# Autodesk Inventor assembly: Pancake_Timing Assy_4 Lanes
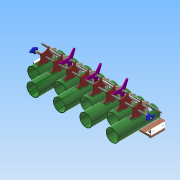
[picture p0: Inventor's stored thumbnail of the model, 180x180]
Saved by Autodesk Inventor 2018.1 (Build 221171000, 171)
## iProperties
Created: 2019-02-11
Part Number: Pancake_Timing Assy_4 Lanes
Document SubType Name: Assembly
Designer: James
Author: James
## Documents named in this file (10)
- C:\Users\admin\Desktop\Ball-Machine\Pancake Sort\Pancake - 4 Lanes\Pancake_Timing Assy_4 Lanes.iam
- C:\Users\admin\Desktop\Ball-Machine\Timing Gate\Nyloc Nut - M4.ipt
- C:\Users\admin\Desktop\Ball-Machine\Timing Gate\Socket Csk Screw - (A2) - M4 x  16.ipt
- C:\Users\admin\Desktop\Ball-Machine\Timing Gate\Socket Cap Screw - Standard - (A2) - M4 x 16.ipt
- C:\Users\admin\Desktop\Ball-Machine\Pancake Sort\Pancake_Angle Bracket.ipt
- C:\Users\admin\Desktop\Ball-Machine\Pancake Sort\Pancake_PVC Pipe.ipt
- C:\Users\admin\Desktop\Ball-Machine\Pancake Sort\Pancake_PVC Pipe Long.ipt
- C:\Users\admin\Desktop\Ball-Machine\Pancake Sort\Pancake - 4 Lanes\Pancake_Timing Assy_Lever Shaft_4 Lanes.iam
- C:\Users\admin\Desktop\Ball-Machine\Pancake Sort\Pancake - 4 Lanes\Pancake_Timing Assy_Star Shaft_4 Lanes.iam
- C:\Users\admin\Desktop\Ball-Machine\Pancake Sort\Pancake - 4 Lanes\Pancake_Timing Backboard_4 Lanes.ipt
## Components (53 placed, 9 different names)
1. Pancake_Timing Backboard_4 Lanes:1 — Angle:2, Tangent:1, Mate:93, Mate:94, Mate:95, Mate:96, Flush:34, Mate:104, Mate:105, Mate:106, Flush:36, Mate:107, Mate:108, Mate:115, Flush:37, Mate:116, Mate:117, Mate:118, Mate:119, Tangent:2, Mate:120, Mate:121
2. Pancake_Timing Assy_Lever Shaft_4 Lanes:1 [sub-assembly] — Flush:96, Flush:97, Flush:31
3. Pancake_Timing Assy_Star Shaft_4 Lanes:1 [sub-assembly] — Flush:94, Angle:2, Flush:93, Flush:95
4. Pancake_Angle Bracket:3 — Mate:104, Mate:105, Mate:106, Flush:36
5. Socket Cap Screw - Standard - (A2) - M4 x 16:7
6. Socket Cap Screw - Standard - (A2) - M4 x 16:8
7. Nyloc Nut - M4:17 — Mate:108
8. Nyloc Nut - M4:18 — Mate:107
9. Pancake_Angle Bracket:4 — Mate:115, Flush:37, Mate:118, Mate:119
10. Nyloc Nut - M4:27 — Mate:117
11. Socket Cap Screw - Standard - (A2) - M4 x 16:9
12. Nyloc Nut - M4:28 — Mate:116
13. Socket Cap Screw - Standard - (A2) - M4 x 16:10
14. Socket Csk Screw - (A2) - M4 x  16:1 — Mate:54, Flush:21, Mate:57, Flush:34
15. Nyloc Nut - M4:2 — Mate:57, Mate:96
16. Socket Csk Screw - (A2) - M4 x  16:2 — Flush:21, Mate:58, Mate:97
17. Nyloc Nut - M4:1 — Mate:58, Mate:95
18. Socket Csk Screw - (A2) - M4 x  16:3
19. Nyloc Nut - M4:19
20. Socket Csk Screw - (A2) - M4 x  16:4
21. Nyloc Nut - M4:20
22. Socket Csk Screw - (A2) - M4 x  16:5
23. Nyloc Nut - M4:21
24. Socket Csk Screw - (A2) - M4 x  16:6
25. Nyloc Nut - M4:22
26. Socket Csk Screw - (A2) - M4 x  16:7
27. Nyloc Nut - M4:23
28. Socket Csk Screw - (A2) - M4 x  16:8
29. Nyloc Nut - M4:24
30. Socket Csk Screw - (A2) - M4 x  16:9
31. Nyloc Nut - M4:25
32. Socket Csk Screw - (A2) - M4 x  16:10
33. Nyloc Nut - M4:26
34. Socket Csk Screw - (A2) - M4 x  16:11
35. Nyloc Nut - M4:29
36. Socket Csk Screw - (A2) - M4 x  16:12
37. Nyloc Nut - M4:30
38. Socket Csk Screw - (A2) - M4 x  16:13
39. Nyloc Nut - M4:31
40. Socket Csk Screw - (A2) - M4 x  16:14
41. Nyloc Nut - M4:32
42. Socket Csk Screw - (A2) - M4 x  16:15
43. Nyloc Nut - M4:33
44. Socket Csk Screw - (A2) - M4 x  16:16
45. Nyloc Nut - M4:34
46. Pancake_PVC Pipe:1 — Angle:1, Mate:54, Tangent:1, Mate:93, Mate:94, Mate:97
47. Pancake_PVC Pipe Long:1 — Tangent:2, Mate:120, Mate:121, Angle:3
48. Pancake_PVC Pipe:2
49. Pancake_PVC Pipe Long:2
50. Pancake_PVC Pipe:3
51. Pancake_PVC Pipe Long:3
52. Pancake_PVC Pipe:4
53. Pancake_PVC Pipe Long:4
## Component patterns: (8 elements, first: Socket Csk Screw - (A2) - M4 x  16:1 + Nyloc Nut - M4:2 + Socket Csk Screw - (A2) - M4 x  16:2 + Nyloc Nut - M4:1), (4 elements, first: Pancake_PVC Pipe:1 + Pancake_PVC Pipe Long:1)
## Relationships (53: Mate 32, Flush 16, Angle 3, Tangent 2)
- Angle:1 (0 deg): Pancake_PVC Pipe:1
- Flush:11 (62.5 mm)
- Flush:12
- Flush:13 (35 mm)
- [Flush]: Pancake_Timing Backboard_4 Lanes:1
- [Flush]: Pancake_Timing Backboard_4 Lanes:1
- [Flush]: Pancake_Timing Backboard_4 Lanes:1
- Mate:54: Socket Csk Screw - (A2) - M4 x  16:1 ↔ Pancake_PVC Pipe:1
- Flush:21: Socket Csk Screw - (A2) - M4 x  16:1 ↔ Socket Csk Screw - (A2) - M4 x  16:2
- Mate:57: Socket Csk Screw - (A2) - M4 x  16:1 ↔ Nyloc Nut - M4:2
- Mate:58: Socket Csk Screw - (A2) - M4 x  16:2 ↔ Nyloc Nut - M4:1
- Flush:96: Pancake_Timing Assy_Lever Shaft_4 Lanes:1
- Flush:97: Pancake_Timing Assy_Lever Shaft_4 Lanes:1
- Flush:31: Pancake_Timing Assy_Lever Shaft_4 Lanes:1
- Flush:94: Pancake_Timing Assy_Star Shaft_4 Lanes:1
- Angle:2 (0 deg): Pancake_Timing Backboard_4 Lanes:1 ↔ Pancake_Timing Assy_Star Shaft_4 Lanes:1
- Flush:93: Pancake_Timing Assy_Star Shaft_4 Lanes:1
- Tangent:1: Pancake_Timing Backboard_4 Lanes:1 ↔ Pancake_PVC Pipe:1
- Mate:93: Pancake_Timing Backboard_4 Lanes:1 ↔ Pancake_PVC Pipe:1
- Mate:94: Pancake_Timing Backboard_4 Lanes:1 ↔ Pancake_PVC Pipe:1
- Mate:95: Pancake_Timing Backboard_4 Lanes:1 ↔ Nyloc Nut - M4:1
- Mate:96: Pancake_Timing Backboard_4 Lanes:1 ↔ Nyloc Nut - M4:2
- Flush:34 (-5 mm): Pancake_Timing Backboard_4 Lanes:1 ↔ Socket Csk Screw - (A2) - M4 x  16:1
- Mate:97: Socket Csk Screw - (A2) - M4 x  16:2 ↔ Pancake_PVC Pipe:1
- [Mate]: Pancake_Angle Bracket:3 ↔ Socket Cap Screw - Standard - (A2) - M4 x 16:8
- [Mate]: Pancake_Angle Bracket:3 ↔ Socket Cap Screw - Standard - (A2) - M4 x 16:8
- [Mate]: Pancake_Angle Bracket:3 ↔ Socket Cap Screw - Standard - (A2) - M4 x 16:7
- [Mate]: Pancake_Angle Bracket:3 ↔ Socket Cap Screw - Standard - (A2) - M4 x 16:7
- [Mate]: Socket Cap Screw - Standard - (A2) - M4 x 16:8 ↔ Nyloc Nut - M4:18
- [Mate]: Socket Cap Screw - Standard - (A2) - M4 x 16:7 ↔ Nyloc Nut - M4:17
- Mate:104: Pancake_Timing Backboard_4 Lanes:1 ↔ Pancake_Angle Bracket:3
- Mate:105: Pancake_Timing Backboard_4 Lanes:1 ↔ Pancake_Angle Bracket:3
- Mate:106: Pancake_Timing Backboard_4 Lanes:1 ↔ Pancake_Angle Bracket:3
- Flush:36: Pancake_Timing Backboard_4 Lanes:1 ↔ Pancake_Angle Bracket:3
- Mate:107: Pancake_Timing Backboard_4 Lanes:1 ↔ Nyloc Nut - M4:18
- Mate:108: Pancake_Timing Backboard_4 Lanes:1 ↔ Nyloc Nut - M4:17
- [Mate]: Pancake_Angle Bracket:4 ↔ Socket Cap Screw - Standard - (A2) - M4 x 16:10
- [Mate]: Pancake_Angle Bracket:4 ↔ Socket Cap Screw - Standard - (A2) - M4 x 16:10
- [Mate]: Pancake_Angle Bracket:4 ↔ Socket Cap Screw - Standard - (A2) - M4 x 16:9
- [Mate]: Pancake_Angle Bracket:4 ↔ Socket Cap Screw - Standard - (A2) - M4 x 16:9
- [Mate]: Nyloc Nut - M4:27 ↔ Socket Cap Screw - Standard - (A2) - M4 x 16:10
- [Mate]: Socket Cap Screw - Standard - (A2) - M4 x 16:9 ↔ Nyloc Nut - M4:28
- Mate:115: Pancake_Timing Backboard_4 Lanes:1 ↔ Pancake_Angle Bracket:4
- Flush:37: Pancake_Timing Backboard_4 Lanes:1 ↔ Pancake_Angle Bracket:4
- Mate:116: Pancake_Timing Backboard_4 Lanes:1 ↔ Nyloc Nut - M4:28
- Mate:117: Pancake_Timing Backboard_4 Lanes:1 ↔ Nyloc Nut - M4:27
- Mate:118: Pancake_Timing Backboard_4 Lanes:1 ↔ Pancake_Angle Bracket:4
- Mate:119: Pancake_Timing Backboard_4 Lanes:1 ↔ Pancake_Angle Bracket:4
- Flush:95: Pancake_Timing Assy_Star Shaft_4 Lanes:1
- Tangent:2: Pancake_Timing Backboard_4 Lanes:1 ↔ Pancake_PVC Pipe Long:1
- Mate:120: Pancake_Timing Backboard_4 Lanes:1 ↔ Pancake_PVC Pipe Long:1
- Mate:121: Pancake_Timing Backboard_4 Lanes:1 ↔ Pancake_PVC Pipe Long:1
- Angle:3 (0 deg): Pancake_PVC Pipe Long:1
## Named parameters: d168_d139_d131 = 0 mm, d169_d140_d132 = 0 mm, d170_d141_d133 = 0 mm, d171_d142_d134 = 0 mm, d172_d149 = 0 mm, d173_d150 = 0 mm, d185_d131 = 0 mm, d186_d132 = 0 mm, d187_d133 = 0 mm, d188_d134 = 0 mm, d189_d137 = 0 mm, d190_d138 = 0 mm
